# Autodesk Inventor assembly: Assemb
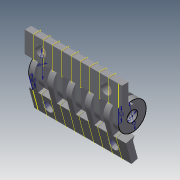
[picture p0: Inventor's stored thumbnail of the model, 180x180]
Saved by Autodesk Inventor 2019 (Build 230136000, 136)
## iProperties
Created: 2020-09-13
Part Number: Assemb
Document SubType Name: Assembly
Designer: giacomo
Author: giacomo
## Documents named in this file (2)
- D:\Hobby\Inventor\Cerniera\Awakening Cerniera\Assemb.iam
- D:\Hobby\Inventor\Cerniera\Awakening Cerniera\parte1.ipt
## Components (2 placed, 1 different names)
1. parte1:1 — Mate:1, Flush:2
2. parte1:2 — Mate:1, Flush:2
## Relationships (2: Mate 1, Flush 1)
- Mate:1: parte1:1 ↔ parte1:2
- Flush:2: parte1:1 ↔ parte1:2
